# Autodesk Inventor assembly: ext
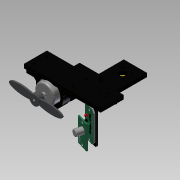
[picture p0: Inventor's stored thumbnail of the model, 180x180]
Saved by Autodesk Inventor 2015 SP1 (Build 190203100, 203)
## iProperties
Created: 2015-02-02
Part Number: ext
Document SubType Name: Assembly
Designer: Rafi Kurnia Putra
Author: Rafi Kurnia Putra
## Documents named in this file (7)
- D:\Dropbox\krpai berkaki trui 2015\ROBUSTA\MEKANIK\ROBUSTA\Assembly Kipas.iam
- D:\Dropbox\krpai berkaki trui 2015\ROBUSTA\MEKANIK\ROBUSTA\Dudukan Kipas.ipt
- D:\Dropbox\krpai berkaki trui 2015\ROBUSTA\MEKANIK\ROBUSTA\Kipas.ipt
- D:\Dropbox\krpai berkaki trui 2015\ROBUSTA\MEKANIK\ROBUSTA\Baling-Baling.ipt
- D:\Dropbox\krpai berkaki trui 2015\ROBUSTA\MEKANIK\ROBUSTA\Dudukan Kipas + TPA.ipt
- D:\Dropbox\krpai berkaki trui 2015\ROBUSTA\MEKANIK\ROBUSTA\Assembly TPA.iam
- D:\Dropbox\krpai berkaki trui 2015\ROBUSTA\MEKANIK\ROBUSTA\Horn Servo.ipt
## Components (6 placed, 6 different names)
1. Dudukan Kipas:1 — Mate:20, Mate:32, Mate:33, Mate:34, Mate:37
2. Kipas:1 — Mate:2, Mate:3, Mate:20, Mate:37
3. Baling-Baling:1 — Mate:2, Mate:3
4. Assembly TPA:1 [sub-assembly] — Mate:29, Mate:35, Mate:36
5. Dudukan Kipas + TPA:1 — Mate:13, Mate:14, Mate:15, Mate:25, Mate:28, Mate:29, Mate:32, Mate:33, Mate:34, Mate:35, Mate:36
6. Horn Servo:1 — Mate:25, Mate:28
## Relationships (15: Mate 15)
- Mate:2: Kipas:1 ↔ Baling-Baling:1
- Mate:3 (4 mm): Kipas:1 ↔ Baling-Baling:1
- Mate:13: Dudukan Kipas + TPA:1
- Mate:14: Dudukan Kipas + TPA:1
- Mate:15: Dudukan Kipas + TPA:1
- Mate:20: Dudukan Kipas:1 ↔ Kipas:1
- Mate:25: Dudukan Kipas + TPA:1 ↔ Horn Servo:1
- Mate:28: Dudukan Kipas + TPA:1 ↔ Horn Servo:1
- Mate:29: Assembly TPA:1 ↔ Dudukan Kipas + TPA:1
- Mate:32: Dudukan Kipas:1 ↔ Dudukan Kipas + TPA:1
- Mate:33: Dudukan Kipas:1 ↔ Dudukan Kipas + TPA:1
- Mate:34: Dudukan Kipas:1 ↔ Dudukan Kipas + TPA:1
- Mate:35: Assembly TPA:1 ↔ Dudukan Kipas + TPA:1
- Mate:36: Assembly TPA:1 ↔ Dudukan Kipas + TPA:1
- Mate:37: Dudukan Kipas:1 ↔ Kipas:1
